# Autodesk Inventor assembly: Button Fixture Assembly
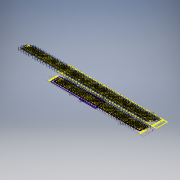
[picture p0: Inventor's stored thumbnail of the model, 180x180]
Saved by Autodesk Inventor 2018.3 (Build 223284000, 284)
## iProperties
Created: 2016-07-07
Part Number: Button Fixture Assembly
Document SubType Name: Assembly
Designer: Sam Clay
Author: Sam Clay
## Documents named in this file (3)
- Z:\enclosure\inventor\Button Fixture Assembly.iam
- Z:\enclosure\inventor\Button Fixture Base.ipt
- Z:\enclosure\inventor\Case Buttons CAM.ipt
## Components (151 placed, 2 different names)
1. Button Fixture Base:1 — Mate:9, Mate:10, Mate:11, Mate:12, Mate:13, Mate:14
2. Case Buttons CAM:9
3. Case Buttons CAM:10
4. Case Buttons CAM:11 — Mate:9
5. Case Buttons CAM:12
6. Case Buttons CAM:41
7. Case Buttons CAM:42 — Mate:13, Mate:14
8. Case Buttons CAM:126
9. Case Buttons CAM:127
10. Case Buttons CAM:128
11. Case Buttons CAM:129
12. Case Buttons CAM:25
13. Case Buttons CAM:26
14. Case Buttons CAM:27
15. Case Buttons CAM:28
16. Case Buttons CAM:53
17. Case Buttons CAM:54
18. Case Buttons CAM:130
19. Case Buttons CAM:131
20. Case Buttons CAM:132
21. Case Buttons CAM:133
22. Case Buttons CAM:90
23. Case Buttons CAM:91
24. Case Buttons CAM:92
25. Case Buttons CAM:93
26. Case Buttons CAM:94
27. Case Buttons CAM:95
28. Case Buttons CAM:134
29. Case Buttons CAM:135
30. Case Buttons CAM:136
31. Case Buttons CAM:137
32. Case Buttons CAM:150
33. Case Buttons CAM:151
34. Case Buttons CAM:152
35. Case Buttons CAM:153
36. Case Buttons CAM:154
37. Case Buttons CAM:155
38. Case Buttons CAM:156
39. Case Buttons CAM:157
40. Case Buttons CAM:158
41. Case Buttons CAM:159
42. Case Buttons CAM:160
43. Case Buttons CAM:161
44. Case Buttons CAM:162
45. Case Buttons CAM:163
46. Case Buttons CAM:164
47. Case Buttons CAM:165
48. Case Buttons CAM:166
49. Case Buttons CAM:167
50. Case Buttons CAM:168
51. Case Buttons CAM:169
52. Case Buttons CAM:170
53. Case Buttons CAM:171
54. Case Buttons CAM:172
55. Case Buttons CAM:173
56. Case Buttons CAM:174
57. Case Buttons CAM:175
58. Case Buttons CAM:176
59. Case Buttons CAM:177
60. Case Buttons CAM:178
61. Case Buttons CAM:179
62. Case Buttons CAM:210
63. Case Buttons CAM:211
64. Case Buttons CAM:212
65. Case Buttons CAM:213
66. Case Buttons CAM:214
67. Case Buttons CAM:215
68. Case Buttons CAM:216
69. Case Buttons CAM:217
70. Case Buttons CAM:218
71. Case Buttons CAM:219
72. Case Buttons CAM:220
73. Case Buttons CAM:221
74. Case Buttons CAM:222
75. Case Buttons CAM:223
76. Case Buttons CAM:224
77. Case Buttons CAM:225
78. Case Buttons CAM:226
79. Case Buttons CAM:227
80. Case Buttons CAM:228
81. Case Buttons CAM:229
82. Case Buttons CAM:230
83. Case Buttons CAM:231
84. Case Buttons CAM:232
85. Case Buttons CAM:233
86. Case Buttons CAM:234
87. Case Buttons CAM:235
88. Case Buttons CAM:236
89. Case Buttons CAM:237
90. Case Buttons CAM:238
91. Case Buttons CAM:239
92. Case Buttons CAM:17 — Mate:10, Mate:11, Mate:12
93. Case Buttons CAM:18
94. Case Buttons CAM:19
95. Case Buttons CAM:20
96. Case Buttons CAM:64
97. Case Buttons CAM:65
98. Case Buttons CAM:138
99. Case Buttons CAM:139
100. Case Buttons CAM:140
101. Case Buttons CAM:141
102. Case Buttons CAM:29
103. Case Buttons CAM:30
104. Case Buttons CAM:31
105. Case Buttons CAM:32
106. Case Buttons CAM:76
107. Case Buttons CAM:77
108. Case Buttons CAM:142
109. Case Buttons CAM:143
110. Case Buttons CAM:144
111. Case Buttons CAM:145
112. Case Buttons CAM:108
113. Case Buttons CAM:109
114. Case Buttons CAM:110
115. Case Buttons CAM:111
116. Case Buttons CAM:112
117. Case Buttons CAM:113
118. Case Buttons CAM:146
119. Case Buttons CAM:147
120. Case Buttons CAM:148
121. Case Buttons CAM:149
122. Case Buttons CAM:180
123. Case Buttons CAM:181
124. Case Buttons CAM:182
125. Case Buttons CAM:183
126. Case Buttons CAM:184
127. Case Buttons CAM:185
128. Case Buttons CAM:186
129. Case Buttons CAM:187
130. Case Buttons CAM:188
131. Case Buttons CAM:189
132. Case Buttons CAM:190
133. Case Buttons CAM:191
134. Case Buttons CAM:192
135. Case Buttons CAM:193
136. Case Buttons CAM:194
137. Case Buttons CAM:195
138. Case Buttons CAM:196
139. Case Buttons CAM:197
140. Case Buttons CAM:198
141. Case Buttons CAM:199
142. Case Buttons CAM:200
143. Case Buttons CAM:201
144. Case Buttons CAM:202
145. Case Buttons CAM:203
146. Case Buttons CAM:204
147. Case Buttons CAM:205
148. Case Buttons CAM:206
149. Case Buttons CAM:207
150. Case Buttons CAM:208
151. Case Buttons CAM:209
## Component patterns: (9 elements), (6 elements), (10 elements, first: Case Buttons CAM:9), Component Pattern 3:2 (10 elements), Component Pattern 3:3 (10 elements), Component Pattern 3:4 (10 elements), Component Pattern 3:5 (10 elements), Component Pattern 3:6 (10 elements), Component Pattern 3:7 (10 elements), Component Pattern 3:8 (10 elements), Component Pattern 3:9 (10 elements), (10 elements, first: Case Buttons CAM:17), Component Pattern 4:2 (10 elements), Component Pattern 4:3 (10 elements), Component Pattern 4:4 (10 elements), Component Pattern 4:5 (10 elements), Component Pattern 4:6 (10 elements)
## Relationships (6: Mate 6)
- Mate:9 (0.762 mm): Button Fixture Base:1 ↔ Case Buttons CAM:11
- Mate:10 (11.43 mm): Button Fixture Base:1 ↔ Case Buttons CAM:17
- Mate:11 (-25.4 mm): Button Fixture Base:1 ↔ Case Buttons CAM:17
- Mate:12 (-38.1 mm): Button Fixture Base:1 ↔ Case Buttons CAM:17
- Mate:13 (5.08 mm): Button Fixture Base:1 ↔ Case Buttons CAM:42
- Mate:14 (1.5875 mm): Button Fixture Base:1 ↔ Case Buttons CAM:42
